# Autodesk Inventor assembly: GP4-100
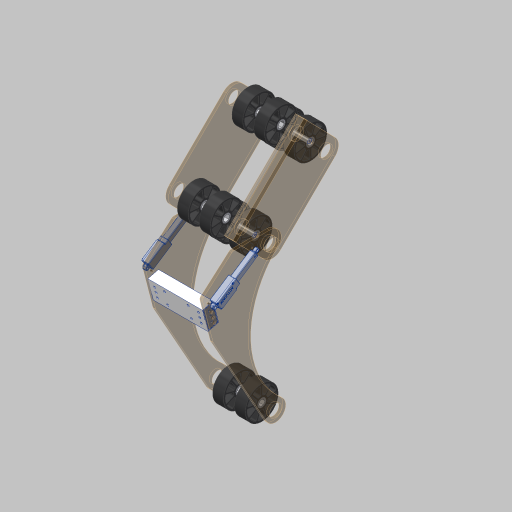
[picture p0: Inventor's stored thumbnail of the model, 512x512]
Saved by Autodesk Inventor 2023.5 (Build 275446000, 446)
## iProperties
Created: 2025-01-28
Part Number: GP4-100
Document SubType Name: Assembly
Designer: slick
Author: slick
## Documents named in this file (10)
- C:\Users\slick\OneDrive\Desktop\2025-ReefScape---CAD\Gripper\GP4\GP4-100.iam
- C:\Users\slick\OneDrive\Desktop\2025-ReefScape---CAD\Gripper\GP4\GP4-001.ipt
- C:\Users\slick\OneDrive\Desktop\2025-ReefScape---CAD\Gripper\GP4\GP4-002.ipt
- C:\Users\slick\OneDrive\Desktop\2025-ReefScape---CAD\Gripper\GP4\GP4-003.ipt
- C:\Users\slick\OneDrive\Desktop\2025-ReefScape---CAD\Gripper\GP4\GP4-003_MIR.ipt
- C:\Users\slick\OneDrive\Desktop\2025-ReefScape---CAD\COMMON PARTS\WHEELS\am-3945 3IN 500Hex Compliant Wheel REV 3.ipt
- C:\Users\slick\OneDrive\Desktop\2025-ReefScape---CAD\Gripper\GP4\GP4-005.ipt
- C:\Users\slick\OneDrive\Desktop\2025-ReefScape---CAD\Gripper\GP4\GP4-006.ipt
- C:\Users\slick\OneDrive\Desktop\2025-ReefScape---CAD\Gripper\GP4\GP4-007.ipt
- C:\Users\slick\OneDrive\Desktop\2025-ReefScape---CAD\COMMON PARTS\Z - STEPS\WCP-0407-Retracted\with movable rod.iam
## Components (21 placed, 9 different names)
1. GP4-001:1 — Insert:1, Insert:2, Mate:2, Mate:6, Mate:11, Mate:14, Mate:26, Mate:27
2. GP4-002:1 — Flush:1, Flush:2, Flush:3, Mate:1, Flush:4, Flush:5
3. GP4-003:1 — Flush:1, Mate:1, Flush:4, Insert:1, Insert:2
4. GP4-003_MIR:1 — Flush:2, Flush:3, Flush:5, Insert:3, Insert:4
5. GP4-001:2 — Insert:3, Insert:4, Mate:7, Mate:10, Mate:12, Mate:13, Mate:23, Mate:24
6. am-3945 3IN 500Hex Compliant Wheel REV 3:1 — Mate:5, Mate:9, Flush:6, Mate:15, Flush:10
7. am-3945 3IN 500Hex Compliant Wheel REV 3:2 — Mate:5, Mate:9, Flush:7, Flush:8
8. am-3945 3IN 500Hex Compliant Wheel REV 3:3 — Mate:7, Mate:8, Flush:8
9. am-3945 3IN 500Hex Compliant Wheel REV 3:4 — Mate:6, Mate:8
10. am-3945 3IN 500Hex Compliant Wheel REV 3:5 — Mate:3, Flush:7, Mate:10
11. am-3945 3IN 500Hex Compliant Wheel REV 3:6 — Mate:2, Mate:3, Flush:6, Flush:9
12. GP4-006:1 — Mate:12, Mate:13, Mate:20, Mate:21, Mate:22, Symmetry:1, Mate:25
13. GP4-005:2 — Mate:11, Mate:14, Mate:15, Mate:22, Symmetry:1, Insert:5, Insert:6, Mate:28
14. am-3945 3IN 500Hex Compliant Wheel REV 3:7 — Mate:20, Flush:10
15. am-3945 3IN 500Hex Compliant Wheel REV 3:8
16. am-3945 3IN 500Hex Compliant Wheel REV 3:9 — Mate:21, Flush:9
17. am-3945 3IN 500Hex Compliant Wheel REV 3:10
18. GP4-007:1 — Insert:6
19. GP4-007:2 — Insert:5
20. with movable rod:1 [sub-assembly] — Mate:23, Mate:24, Mate:25
21. with movable rod:2 [sub-assembly] — Mate:26, Mate:27, Mate:28
## Relationships (44: Mate 27, Flush 10, Insert 6, Symmetry 1)
- Flush:1: GP4-002:1 ↔ GP4-003:1
- Flush:2: GP4-002:1 ↔ GP4-003_MIR:1
- Flush:3: GP4-002:1 ↔ GP4-003_MIR:1
- Mate:1: GP4-002:1 ↔ GP4-003:1
- Flush:4: GP4-002:1 ↔ GP4-003:1
- Flush:5: GP4-002:1 ↔ GP4-003_MIR:1
- Insert:1: GP4-001:1 ↔ GP4-003:1
- Insert:2: GP4-001:1 ↔ GP4-003:1
- Insert:3: GP4-003_MIR:1 ↔ GP4-001:2
- Insert:4: GP4-003_MIR:1 ↔ GP4-001:2
- Mate:2: GP4-001:1 ↔ am-3945 3IN 500Hex Compliant Wheel REV 3:6
- Mate:3: am-3945 3IN 500Hex Compliant Wheel REV 3:5 ↔ am-3945 3IN 500Hex Compliant Wheel REV 3:6
- Mate:5: am-3945 3IN 500Hex Compliant Wheel REV 3:1 ↔ am-3945 3IN 500Hex Compliant Wheel REV 3:2
- Mate:6: GP4-001:1 ↔ am-3945 3IN 500Hex Compliant Wheel REV 3:4
- Mate:7: GP4-001:2 ↔ am-3945 3IN 500Hex Compliant Wheel REV 3:3
- Mate:8 (25.4 mm): am-3945 3IN 500Hex Compliant Wheel REV 3:3 ↔ am-3945 3IN 500Hex Compliant Wheel REV 3:4
- Mate:9 (25.4 mm): am-3945 3IN 500Hex Compliant Wheel REV 3:1 ↔ am-3945 3IN 500Hex Compliant Wheel REV 3:2
- Flush:6: am-3945 3IN 500Hex Compliant Wheel REV 3:1 ↔ am-3945 3IN 500Hex Compliant Wheel REV 3:6
- Flush:7: am-3945 3IN 500Hex Compliant Wheel REV 3:2 ↔ am-3945 3IN 500Hex Compliant Wheel REV 3:5
- Mate:10 (25.4 mm): GP4-001:2 ↔ am-3945 3IN 500Hex Compliant Wheel REV 3:5
- Flush:8: am-3945 3IN 500Hex Compliant Wheel REV 3:2 ↔ am-3945 3IN 500Hex Compliant Wheel REV 3:3
- Mate:11: GP4-001:1 ↔ GP4-005:2
- Mate:12: GP4-001:2 ↔ GP4-006:1
- Mate:13: GP4-001:2 ↔ GP4-006:1
- Mate:14: GP4-001:1 ↔ GP4-005:2
- Mate:15: am-3945 3IN 500Hex Compliant Wheel REV 3:1 ↔ GP4-005:2
- [Mate]: am-3945 3IN 500Hex Compliant Wheel REV 3:7 ↔ am-3945 3IN 500Hex Compliant Wheel REV 3:8
- [Mate] (25.4 mm): am-3945 3IN 500Hex Compliant Wheel REV 3:7 ↔ am-3945 3IN 500Hex Compliant Wheel REV 3:8
- [Mate]: am-3945 3IN 500Hex Compliant Wheel REV 3:9 ↔ am-3945 3IN 500Hex Compliant Wheel REV 3:10
- [Mate] (25.4 mm): am-3945 3IN 500Hex Compliant Wheel REV 3:9 ↔ am-3945 3IN 500Hex Compliant Wheel REV 3:10
- Mate:20: GP4-006:1 ↔ am-3945 3IN 500Hex Compliant Wheel REV 3:7
- Mate:21: GP4-006:1 ↔ am-3945 3IN 500Hex Compliant Wheel REV 3:9
- Flush:9: am-3945 3IN 500Hex Compliant Wheel REV 3:6 ↔ am-3945 3IN 500Hex Compliant Wheel REV 3:9
- Flush:10: am-3945 3IN 500Hex Compliant Wheel REV 3:1 ↔ am-3945 3IN 500Hex Compliant Wheel REV 3:7
- Mate:22: GP4-006:1 ↔ GP4-005:2
- Symmetry:1: GP4-006:1 ↔ GP4-005:2
- Insert:5: GP4-005:2 ↔ GP4-007:2
- Insert:6: GP4-005:2 ↔ GP4-007:1
- Mate:23: GP4-001:2 ↔ with movable rod:1
- Mate:24: GP4-001:2 ↔ with movable rod:1
- Mate:25: GP4-006:1 ↔ with movable rod:1
- Mate:26: GP4-001:1 ↔ with movable rod:2
- Mate:27: GP4-001:1 ↔ with movable rod:2
- Mate:28: GP4-005:2 ↔ with movable rod:2
## Named parameters: d53_d33 = 0 mm, d54_d37 = 25.4 mm, d55_d33 = 0 mm, d56_d37 = 25.4 mm
